# Autodesk Inventor assembly: Chassis Assembly 26x28 Version
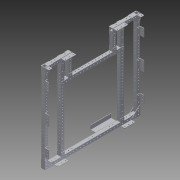
[picture p0: Inventor's stored thumbnail of the model, 180x180]
Saved by Autodesk Inventor 2013 (Build 170138000, 138)
## iProperties
Created: 2013-01-06
Part Number: Chassis Assembly 26x28 Version
Document SubType Name: Assembly
Designer: Moses
Mass: 3880.88 g
Surface Area: 9738.61 cm^2
Volume: 1432.06 cm^3
Density: 2.71 g/cm^3
Author: Moses
## Documents named in this file (17)
- C:\Users\Moses\Documents\GitHub\frc2013CAD\Chassis\Chassis Assembly 26x28 Version\Chassis Assembly 26x28 Version.iam
- C:\Users\Moses\Documents\GitHub\frc2013CAD\Chassis\Chassis V1.500 Part3-mirror.ipt
- C:\Users\Moses\Documents\GitHub\frc2013CAD\Chassis\Chassis V1.500 Part8.ipt
- C:\Users\Moses\Documents\GitHub\frc2013CAD\Chassis\Chassis V1.500 Part7.ipt
- C:\Users\Moses\Documents\GitHub\frc2013CAD\Chassis\Chassis V1.500 Part2.ipt
- C:\Users\Moses\Documents\GitHub\frc2013CAD\Chassis\Chassis V1.500 Part3.ipt
- C:\Users\Moses\Documents\GitHub\frc2013CAD\Chassis\Chassis Connector Plate V1.500.ipt
- C:\Users\Moses\Documents\GitHub\frc2013CAD\Chassis\Chassis Corner Plate V1.500.ipt
- C:\Users\Moses\Documents\GitHub\frc2013CAD\Chassis\Chassis Assembly 26x28 Version\Chassis Part4 (26x28).ipt
- C:\Users\Moses\Documents\GitHub\frc2013CAD\Chassis\Chassis Assembly 26x28 Version\Chassis Part1 (26x28).ipt
- C:\Users\Moses\Documents\GitHub\frc2013CAD\Chassis\Chassis Assembly 26x28 Version\Chassis Battery Mount Part1.ipt
- C:\Users\Moses\Documents\GitHub\frc2013CAD\Chassis\Chassis Assembly 26x28 Version\Chassis Bumper Mount - side - center.ipt
- C:\Users\Moses\Documents\GitHub\frc2013CAD\Chassis\Chassis Assembly 26x28 Version\Chassis Bumper Mount - side - ends.ipt
- C:\Users\Moses\Documents\GitHub\frc2013CAD\Chassis\Chassis Assembly 26x28 Version\Chassis Bumper Mount - front - end.ipt
- C:\Users\Moses\Documents\GitHub\frc2013CAD\Chassis\Chassis Assembly 26x28 Version\Chassis Bumper Mount - front - end - large.ipt
- C:\Users\Moses\Documents\GitHub\frc2013CAD\Chassis\Chassis Assembly 26x28 Version\Chassis Bumper Mount - back.ipt
- C:\Users\Moses\Documents\GitHub\frc2013CAD\Chassis\Chassis Assembly 26x28 Version\Chassis Bumper Mount - back - mirror.ipt
## Components (45 placed, 16 different names)
1. Chassis Part1 (26x28):1 — Mate:2, Flush:3, Flush:4, Flush:12, Mate:6, Flush:21, Flush:22, Mate:14, Flush:23, Flush:24, Mate:15, Flush:26, Mate:16, Flush:27, Flush:28, Flush:25, Mate:82, Mate:83, Mate:84, Mate:91, Mate:92, Mate:93, Mate:94, Mate:95, Mate:96
2. Chassis Part1 (26x28):2 — Mate:3, Flush:5, Flush:6, Flush:10, Mate:5, Flush:17, Mate:17, Flush:29, Flush:30, Mate:18, Flush:31, Flush:32, Mate:19, Flush:33, Flush:34, Mate:20, Flush:35, Flush:36, Mate:79, Mate:80, Mate:81, Mate:85, Mate:86, Mate:87, Mate:88, Mate:89, Mate:90, Mate:111
3. Chassis V1.500 Part2:1 — Mate:2, Flush:3, Flush:4, Mate:3, Flush:5, Flush:6, Mate:8, Mate:9, Flush:15, Flush:16, Mate:36, Mate:37, Mate:39, Mate:40, Mate:76, Mate:77, Mate:78, Mate:100, Mate:102, Mate:106, Mate:108
4. Chassis Part4 (26x28):1 — Flush:10, Mate:4, Flush:13, Mate:8, Flush:16, Mate:35, Mate:38, Mate:45, Flush:37, Mate:101, Mate:117
5. Chassis Part4 (26x28):2 — Flush:12, Flush:14, Mate:7, Mate:9, Flush:15, Mate:41, Mate:44, Mate:107, Mate:120
6. Chassis V1.500 Part3-mirror:1 — Mate:4, Mate:5, Flush:13, Mate:33, Mate:34, Flush:38, Mate:54, Flush:43, Flush:44, Mate:61, Mate:115
7. Chassis V1.500 Part3:1 — Mate:6, Flush:14, Mate:7, Mate:13, Mate:42, Mate:43, Mate:55, Flush:45, Flush:46, Mate:64, Mate:118
8. Chassis Corner Plate V1.500:1 — Flush:21, Mate:13, Flush:22
9. Chassis Corner Plate V1.500:2 — Mate:14, Flush:23, Flush:24, Mate:112, Mate:113, Mate:114
10. Chassis Corner Plate V1.500:3 — Mate:15, Flush:25, Flush:26
11. Chassis Corner Plate V1.500:4 — Mate:16, Flush:27, Flush:28
12. Chassis Corner Plate V1.500:5 — Mate:17, Flush:29, Flush:30
13. Chassis Corner Plate V1.500:6 — Mate:18, Flush:31, Flush:32
14. Chassis Corner Plate V1.500:7 — Mate:19, Flush:33, Flush:34
15. Chassis Corner Plate V1.500:8 — Mate:20, Flush:35, Flush:36, Mate:109, Mate:110
16. Chassis Connector Plate V1.500:5 — Mate:33, Mate:34, Mate:35
17. Chassis Connector Plate V1.500:6 — Mate:36, Mate:37, Mate:38
18. Chassis Connector Plate V1.500:7 — Mate:39, Mate:40, Mate:41
19. Chassis Connector Plate V1.500:8 — Mate:42, Mate:43, Mate:44
20. Chassis V1.500 Part7:1 — Mate:45, Flush:37, Flush:38, Mate:46, Mate:47, Flush:39, Mate:48, Mate:49, Flush:40, Mate:50, Mate:51, Flush:41, Mate:52, Mate:53, Flush:42
21. Chassis Connector Plate V1.500:9 — Mate:52, Mate:53, Flush:42
22. Chassis Connector Plate V1.500:10 — Mate:50, Mate:51, Flush:41
23. Chassis Connector Plate V1.500:11 — Mate:48, Mate:49, Flush:40
24. Chassis Connector Plate V1.500:12 — Mate:46, Mate:47, Flush:39
25. Chassis V1.500 Part8:1 — Mate:54, Flush:43, Flush:44, Mate:59, Mate:60, Mate:68, Mate:69, Flush:47, Mate:70, Mate:71, Flush:48, Mate:116
26. Chassis V1.500 Part8:2 — Mate:55, Flush:45, Flush:46, Mate:62, Mate:63, Mate:72, Mate:73, Mate:74, Mate:75, Flush:49, Flush:50, Mate:119
27. Chassis Connector Plate V1.500:14 — Mate:59, Mate:60, Mate:61
28. Chassis Connector Plate V1.500:16 — Mate:62, Mate:63, Mate:64
29. Chassis Connector Plate V1.500:17 — Mate:68, Mate:69, Flush:47
30. Chassis Connector Plate V1.500:18 — Mate:70, Mate:71, Flush:48
31. Chassis Connector Plate V1.500:19 — Mate:72, Mate:73, Flush:50
32. Chassis Connector Plate V1.500:20 — Mate:74, Mate:75, Flush:49
33. Chassis Battery Mount Part1:1 — Mate:76, Mate:77, Mate:78
34. Chassis Bumper Mount - side - center:1 — Mate:79, Mate:80, Mate:81
35. Chassis Bumper Mount - side - center:2 — Mate:82, Mate:83, Mate:84
36. Chassis Bumper Mount - side - ends:1 — Mate:85, Mate:86, Mate:87
37. Chassis Bumper Mount - side - ends:2 — Mate:88, Mate:89, Mate:90
38. Chassis Bumper Mount - side - ends:3 — Mate:91, Mate:92, Mate:93
39. Chassis Bumper Mount - side - ends:4 — Mate:94, Mate:95, Mate:96
40. Chassis Bumper Mount - back:1 — Mate:100, Mate:101, Mate:102
41. Chassis Bumper Mount - back - mirror:1 — Mate:106, Mate:107, Mate:108
42. Chassis Bumper Mount - front - end:1 — Mate:109, Mate:110, Mate:111
43. Chassis Bumper Mount - front - end:2 — Mate:112, Mate:113, Mate:114
44. Chassis Bumper Mount - front - end - large:1 — Mate:115, Mate:116, Mate:117
45. Chassis Bumper Mount - front - end - large:2 — Mate:118, Mate:119, Mate:120
## Relationships (133: Mate 92, Flush 41)
- Mate:2: Chassis Part1 (26x28):1 ↔ Chassis V1.500 Part2:1
- Flush:3: Chassis Part1 (26x28):1 ↔ Chassis V1.500 Part2:1
- Flush:4: Chassis Part1 (26x28):1 ↔ Chassis V1.500 Part2:1
- Mate:3: Chassis Part1 (26x28):2 ↔ Chassis V1.500 Part2:1
- Flush:5: Chassis Part1 (26x28):2 ↔ Chassis V1.500 Part2:1
- Flush:6: Chassis Part1 (26x28):2 ↔ Chassis V1.500 Part2:1
- Flush:10 (-120.65 mm): Chassis Part1 (26x28):2 ↔ Chassis Part4 (26x28):1
- Flush:12 (-120.65 mm): Chassis Part1 (26x28):1 ↔ Chassis Part4 (26x28):2
- Mate:4: Chassis Part4 (26x28):1 ↔ Chassis V1.500 Part3-mirror:1
- Mate:5: Chassis Part1 (26x28):2 ↔ Chassis V1.500 Part3-mirror:1
- Flush:13: Chassis Part4 (26x28):1 ↔ Chassis V1.500 Part3-mirror:1
- Mate:6: Chassis Part1 (26x28):1 ↔ Chassis V1.500 Part3:1
- Flush:14: Chassis Part4 (26x28):2 ↔ Chassis V1.500 Part3:1
- Mate:7: Chassis Part4 (26x28):2 ↔ Chassis V1.500 Part3:1
- Mate:8: Chassis V1.500 Part2:1 ↔ Chassis Part4 (26x28):1
- Mate:9: Chassis V1.500 Part2:1 ↔ Chassis Part4 (26x28):2
- Flush:15: Chassis V1.500 Part2:1 ↔ Chassis Part4 (26x28):2
- Flush:16: Chassis V1.500 Part2:1 ↔ Chassis Part4 (26x28):1
- Flush:17 (330.2 mm): Chassis Part1 (26x28):2
- Flush:21: Chassis Part1 (26x28):1 ↔ Chassis Corner Plate V1.500:1
- Mate:13: Chassis V1.500 Part3:1 ↔ Chassis Corner Plate V1.500:1
- Flush:22: Chassis Part1 (26x28):1 ↔ Chassis Corner Plate V1.500:1
- Mate:14: Chassis Part1 (26x28):1 ↔ Chassis Corner Plate V1.500:2
- Flush:23: Chassis Part1 (26x28):1 ↔ Chassis Corner Plate V1.500:2
- Flush:24: Chassis Part1 (26x28):1 ↔ Chassis Corner Plate V1.500:2
- Mate:15: Chassis Part1 (26x28):1 ↔ Chassis Corner Plate V1.500:3
- Flush:25: Chassis Part1 (26x28):1 ↔ Chassis Corner Plate V1.500:3
- Flush:26: Chassis Part1 (26x28):1 ↔ Chassis Corner Plate V1.500:3
- Mate:16: Chassis Part1 (26x28):1 ↔ Chassis Corner Plate V1.500:4
- Flush:27: Chassis Part1 (26x28):1 ↔ Chassis Corner Plate V1.500:4
- Flush:28: Chassis Part1 (26x28):1 ↔ Chassis Corner Plate V1.500:4
- Mate:17: Chassis Part1 (26x28):2 ↔ Chassis Corner Plate V1.500:5
- Flush:29: Chassis Part1 (26x28):2 ↔ Chassis Corner Plate V1.500:5
- Flush:30: Chassis Part1 (26x28):2 ↔ Chassis Corner Plate V1.500:5
- Mate:18: Chassis Part1 (26x28):2 ↔ Chassis Corner Plate V1.500:6
- Flush:31: Chassis Part1 (26x28):2 ↔ Chassis Corner Plate V1.500:6
- Flush:32: Chassis Part1 (26x28):2 ↔ Chassis Corner Plate V1.500:6
- Mate:19: Chassis Part1 (26x28):2 ↔ Chassis Corner Plate V1.500:7
- Flush:33: Chassis Part1 (26x28):2 ↔ Chassis Corner Plate V1.500:7
- Flush:34: Chassis Part1 (26x28):2 ↔ Chassis Corner Plate V1.500:7
- Mate:20: Chassis Part1 (26x28):2 ↔ Chassis Corner Plate V1.500:8
- Flush:35: Chassis Part1 (26x28):2 ↔ Chassis Corner Plate V1.500:8
- Flush:36: Chassis Part1 (26x28):2 ↔ Chassis Corner Plate V1.500:8
- Mate:33: Chassis V1.500 Part3-mirror:1 ↔ Chassis Connector Plate V1.500:5
- Mate:34: Chassis V1.500 Part3-mirror:1 ↔ Chassis Connector Plate V1.500:5
- Mate:35: Chassis Part4 (26x28):1 ↔ Chassis Connector Plate V1.500:5
- Mate:36: Chassis V1.500 Part2:1 ↔ Chassis Connector Plate V1.500:6
- Mate:37: Chassis V1.500 Part2:1 ↔ Chassis Connector Plate V1.500:6
- Mate:38: Chassis Part4 (26x28):1 ↔ Chassis Connector Plate V1.500:6
- Mate:39: Chassis V1.500 Part2:1 ↔ Chassis Connector Plate V1.500:7
- Mate:40: Chassis V1.500 Part2:1 ↔ Chassis Connector Plate V1.500:7
- Mate:41: Chassis Part4 (26x28):2 ↔ Chassis Connector Plate V1.500:7
- Mate:42: Chassis V1.500 Part3:1 ↔ Chassis Connector Plate V1.500:8
- Mate:43: Chassis V1.500 Part3:1 ↔ Chassis Connector Plate V1.500:8
- Mate:44: Chassis Part4 (26x28):2 ↔ Chassis Connector Plate V1.500:8
- Mate:45: Chassis Part4 (26x28):1 ↔ Chassis V1.500 Part7:1
- Flush:37: Chassis Part4 (26x28):1 ↔ Chassis V1.500 Part7:1
- Flush:38 (-152.4 mm): Chassis V1.500 Part3-mirror:1 ↔ Chassis V1.500 Part7:1
- Mate:46: Chassis V1.500 Part7:1 ↔ Chassis Connector Plate V1.500:12
- Mate:47: Chassis V1.500 Part7:1 ↔ Chassis Connector Plate V1.500:12
- Flush:39: Chassis V1.500 Part7:1 ↔ Chassis Connector Plate V1.500:12
- Mate:48: Chassis V1.500 Part7:1 ↔ Chassis Connector Plate V1.500:11
- Mate:49: Chassis V1.500 Part7:1 ↔ Chassis Connector Plate V1.500:11
- Flush:40: Chassis V1.500 Part7:1 ↔ Chassis Connector Plate V1.500:11
- Mate:50: Chassis V1.500 Part7:1 ↔ Chassis Connector Plate V1.500:10
- Mate:51: Chassis V1.500 Part7:1 ↔ Chassis Connector Plate V1.500:10
- Flush:41: Chassis V1.500 Part7:1 ↔ Chassis Connector Plate V1.500:10
- Mate:52: Chassis V1.500 Part7:1 ↔ Chassis Connector Plate V1.500:9
- Mate:53: Chassis V1.500 Part7:1 ↔ Chassis Connector Plate V1.500:9
- Flush:42: Chassis V1.500 Part7:1 ↔ Chassis Connector Plate V1.500:9
- Mate:54: Chassis V1.500 Part3-mirror:1 ↔ Chassis V1.500 Part8:1
- Flush:43: Chassis V1.500 Part3-mirror:1 ↔ Chassis V1.500 Part8:1
- Flush:44: Chassis V1.500 Part3-mirror:1 ↔ Chassis V1.500 Part8:1
- Mate:55: Chassis V1.500 Part3:1 ↔ Chassis V1.500 Part8:2
- Flush:45: Chassis V1.500 Part3:1 ↔ Chassis V1.500 Part8:2
- Flush:46: Chassis V1.500 Part3:1 ↔ Chassis V1.500 Part8:2
- Mate:59: Chassis V1.500 Part8:1 ↔ Chassis Connector Plate V1.500:14
- Mate:60: Chassis V1.500 Part8:1 ↔ Chassis Connector Plate V1.500:14
- Mate:61: Chassis V1.500 Part3-mirror:1 ↔ Chassis Connector Plate V1.500:14
- Mate:62: Chassis V1.500 Part8:2 ↔ Chassis Connector Plate V1.500:16
- Mate:63: Chassis V1.500 Part8:2 ↔ Chassis Connector Plate V1.500:16
- Mate:64: Chassis V1.500 Part3:1 ↔ Chassis Connector Plate V1.500:16
- Mate:68: Chassis V1.500 Part8:1 ↔ Chassis Connector Plate V1.500:17
- Mate:69: Chassis V1.500 Part8:1 ↔ Chassis Connector Plate V1.500:17
- Flush:47: Chassis V1.500 Part8:1 ↔ Chassis Connector Plate V1.500:17
- Mate:70: Chassis V1.500 Part8:1 ↔ Chassis Connector Plate V1.500:18
- Mate:71: Chassis V1.500 Part8:1 ↔ Chassis Connector Plate V1.500:18
- Flush:48: Chassis V1.500 Part8:1 ↔ Chassis Connector Plate V1.500:18
- Mate:72: Chassis V1.500 Part8:2 ↔ Chassis Connector Plate V1.500:19
- Mate:73: Chassis V1.500 Part8:2 ↔ Chassis Connector Plate V1.500:19
- Mate:74: Chassis V1.500 Part8:2 ↔ Chassis Connector Plate V1.500:20
- Mate:75: Chassis V1.500 Part8:2 ↔ Chassis Connector Plate V1.500:20
- Flush:49: Chassis V1.500 Part8:2 ↔ Chassis Connector Plate V1.500:20
- Flush:50: Chassis V1.500 Part8:2 ↔ Chassis Connector Plate V1.500:19
- Mate:76: Chassis V1.500 Part2:1 ↔ Chassis Battery Mount Part1:1
- Mate:77: Chassis V1.500 Part2:1 ↔ Chassis Battery Mount Part1:1
- Mate:78: Chassis V1.500 Part2:1 ↔ Chassis Battery Mount Part1:1
- Mate:79: Chassis Part1 (26x28):2 ↔ Chassis Bumper Mount - side - center:1
- Mate:80: Chassis Part1 (26x28):2 ↔ Chassis Bumper Mount - side - center:1
- Mate:81: Chassis Part1 (26x28):2 ↔ Chassis Bumper Mount - side - center:1
- Mate:82: Chassis Part1 (26x28):1 ↔ Chassis Bumper Mount - side - center:2
- Mate:83: Chassis Part1 (26x28):1 ↔ Chassis Bumper Mount - side - center:2
- Mate:84: Chassis Part1 (26x28):1 ↔ Chassis Bumper Mount - side - center:2
- Mate:85: Chassis Part1 (26x28):2 ↔ Chassis Bumper Mount - side - ends:1
- Mate:86: Chassis Part1 (26x28):2 ↔ Chassis Bumper Mount - side - ends:1
- Mate:87: Chassis Part1 (26x28):2 ↔ Chassis Bumper Mount - side - ends:1
- Mate:88: Chassis Part1 (26x28):2 ↔ Chassis Bumper Mount - side - ends:2
- Mate:89: Chassis Part1 (26x28):2 ↔ Chassis Bumper Mount - side - ends:2
- Mate:90: Chassis Part1 (26x28):2 ↔ Chassis Bumper Mount - side - ends:2
- Mate:91: Chassis Part1 (26x28):1 ↔ Chassis Bumper Mount - side - ends:3
- Mate:92: Chassis Part1 (26x28):1 ↔ Chassis Bumper Mount - side - ends:3
- Mate:93: Chassis Part1 (26x28):1 ↔ Chassis Bumper Mount - side - ends:3
- Mate:94: Chassis Part1 (26x28):1 ↔ Chassis Bumper Mount - side - ends:4
- Mate:95: Chassis Part1 (26x28):1 ↔ Chassis Bumper Mount - side - ends:4
- Mate:96: Chassis Part1 (26x28):1 ↔ Chassis Bumper Mount - side - ends:4
- Mate:100: Chassis V1.500 Part2:1 ↔ Chassis Bumper Mount - back:1
- Mate:101: Chassis Part4 (26x28):1 ↔ Chassis Bumper Mount - back:1
- Mate:102: Chassis V1.500 Part2:1 ↔ Chassis Bumper Mount - back:1
- Mate:106: Chassis V1.500 Part2:1 ↔ Chassis Bumper Mount - back - mirror:1
- Mate:107: Chassis Part4 (26x28):2 ↔ Chassis Bumper Mount - back - mirror:1
- Mate:108: Chassis V1.500 Part2:1 ↔ Chassis Bumper Mount - back - mirror:1
- Mate:109: Chassis Corner Plate V1.500:8 ↔ Chassis Bumper Mount - front - end:1
- Mate:110: Chassis Corner Plate V1.500:8 ↔ Chassis Bumper Mount - front - end:1
- Mate:111: Chassis Part1 (26x28):2 ↔ Chassis Bumper Mount - front - end:1
- Mate:112: Chassis Corner Plate V1.500:2 ↔ Chassis Bumper Mount - front - end:2
- Mate:113: Chassis Corner Plate V1.500:2 ↔ Chassis Bumper Mount - front - end:2
- Mate:114: Chassis Corner Plate V1.500:2 ↔ Chassis Bumper Mount - front - end:2
- Mate:115: Chassis V1.500 Part3-mirror:1 ↔ Chassis Bumper Mount - front - end - large:1
- Mate:116: Chassis V1.500 Part8:1 ↔ Chassis Bumper Mount - front - end - large:1
- Mate:117: Chassis Part4 (26x28):1 ↔ Chassis Bumper Mount - front - end - large:1
- Mate:118: Chassis V1.500 Part3:1 ↔ Chassis Bumper Mount - front - end - large:2
- Mate:119: Chassis V1.500 Part8:2 ↔ Chassis Bumper Mount - front - end - large:2
- Mate:120: Chassis Part4 (26x28):2 ↔ Chassis Bumper Mount - front - end - large:2
